# Autodesk Inventor assembly: Муфта двигателя
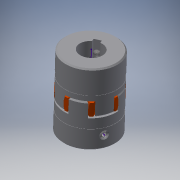
[picture p0: Inventor's stored thumbnail of the model, 180x180]
Saved by Autodesk Inventor 2016 (Build 200138000, 138)
## iProperties
Created: 2021-04-30
Part Number: Муфта двигателя
Material: Типовые
Document SubType Name: Assembly
Designer: Лол
Author: Лол
## Documents named in this file (6)
- C:\Users\Лол\Documents\Inventor\course_work\Муфта двигателя.iam
- C:\Users\Лол\Documents\Inventor\course_work\Муфта железка мотора 38мм.ipt
- C:\Users\Лол\Documents\Inventor\course_work\Муфта железка редуктора 28мм.ipt
- C:\Users\Лол\Documents\Inventor\course_work\Муфта резинка 28мм.ipt
- C:\Users\Лол\Documents\Inventor\course_work\AS 1421 - M8x10 конический.ipt
- C:\Users\Лол\Documents\Inventor\course_work\AS 1421 - M8x16 конический.ipt
## Components (5 placed, 5 different names)
1. Муфта железка мотора 38мм:1 — Совмещение:1, Совмещение:2, Совмещение:4, Угол:2, Совмещение:5, Заподлицо:1
2. Муфта резинка 28мм:1 — Совмещение:1, Совмещение:2, Совмещение:3, Угол:1
3. Муфта железка редуктора 28мм:1 — Совмещение:3, Совмещение:4, Угол:1, Угол:2, Совмещение:6, Заподлицо:2
4. AS 1421 - M8x10 конический:1 — Совмещение:5, Заподлицо:1
5. AS 1421 - M8x16 конический:1 — Совмещение:6, Заподлицо:2
## Relationships (10: Mate 6, Angle 2, Flush 2)
- Совмещение:1 [Mate]: Муфта железка мотора 38мм:1 ↔ Муфта резинка 28мм:1
- Совмещение:2 [Mate]: Муфта железка мотора 38мм:1 ↔ Муфта резинка 28мм:1
- Совмещение:3 [Mate]: Муфта резинка 28мм:1 ↔ Муфта железка редуктора 28мм:1
- Совмещение:4 [Mate]: Муфта железка мотора 38мм:1 ↔ Муфта железка редуктора 28мм:1
- Угол:1 [Angle] (22.5 deg): Муфта резинка 28мм:1 ↔ Муфта железка редуктора 28мм:1
- Угол:2 [Angle] (45 deg): Муфта железка мотора 38мм:1 ↔ Муфта железка редуктора 28мм:1
- Совмещение:5 [Mate]: Муфта железка мотора 38мм:1 ↔ AS 1421 - M8x10 конический:1
- Заподлицо:1 [Flush] (-0.3 mm): Муфта железка мотора 38мм:1 ↔ AS 1421 - M8x10 конический:1
- Совмещение:6 [Mate]: Муфта железка редуктора 28мм:1 ↔ AS 1421 - M8x16 конический:1
- Заподлицо:2 [Flush] (-1 mm): Муфта железка редуктора 28мм:1 ↔ AS 1421 - M8x16 конический:1
